# Autodesk Inventor assembly: Demonstrator
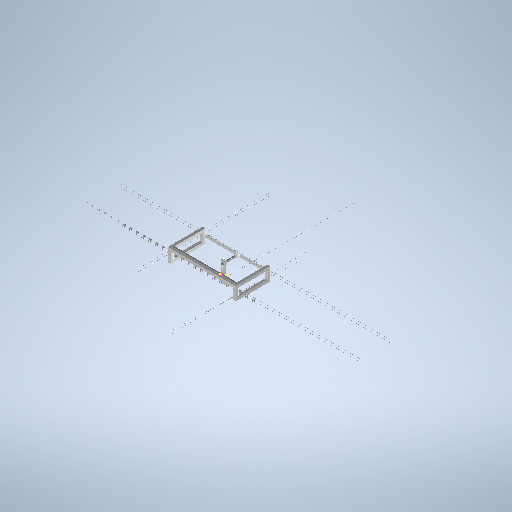
[picture p0: Inventor's stored thumbnail of the model, 512x512]
Saved by Autodesk Inventor 2025 (Build 290162010, 162A)
## iProperties
Created: 2024-11-07
Part Number: Demonstrator
Document SubType Name: Assembly
Designer: Admin
Mass: 19761.8 g
Surface Area: 23870.2 cm^2
Volume: 8041.77 cm^3
Density: 2.4574 g/cm^3
dummerWinkel: 1.5
Author: Admin
## Documents named in this file (23)
- C:\Users\Admin\Documents\Inventor\Krandemonstrator\Demonstrator.iam
- C:\Users\Admin\Documents\Inventor\Krandemonstrator\Träger.ipt
- C:\Users\Admin\Documents\Inventor\Content Center Files\R2025\de-DE\GB 798-88\Eye bolt GB 798 M4 x 20.ipt
- C:\Users\Admin\Documents\Inventor\Content Center Files\R2025\de-DE\AS 1112 (2)\AS 1112 - M4  Typ 5.ipt
- C:\Users\Admin\Documents\Inventor\Krandemonstrator\MontageAufnahmeLO.ipt
- C:\Users\Admin\Documents\Inventor\Krandemonstrator\MontageAufnahmeLOV.ipt
- C:\Users\Admin\Documents\Inventor\Krandemonstrator\FrameSide.ipt
- C:\Users\Admin\Documents\Inventor\Krandemonstrator\FrameSideR.ipt
- C:\Users\Admin\Documents\Inventor\Content Center Files\R2025\de-DE\AS 1427(03)\AS 1427 - M2 x 6(1).ipt
- C:\Users\Admin\Documents\Inventor\Krandemonstrator\Katze.iam
- C:\Users\Admin\Documents\Inventor\Krandemonstrator\UmlenkrolleHalterEinfach.iam
- C:\Users\Admin\Documents\Inventor\Krandemonstrator\SeilStange1m.ipt
- C:\Users\Admin\Documents\Inventor\Krandemonstrator\RollenhalterU.ipt
- C:\Users\Admin\Documents\Inventor\Krandemonstrator\UmlenkrolleHalterDoppelt.iam
- C:\Users\Admin\Documents\Inventor\Krandemonstrator\SeilatrappeHalter.ipt
- C:\Users\Admin\Documents\Inventor\Krandemonstrator\UmlenkrolleHalterDoppeltAngle.iam
- C:\Users\Admin\Documents\Inventor\Krandemonstrator\UmlenkrolleHalterEinfachAngle.iam
- C:\Users\Admin\Documents\Inventor\Krandemonstrator\UmlenkrolleHalterEinfachAngleB.iam
- C:\Users\Admin\Documents\Inventor\Krandemonstrator\seilatrappeHalterMini.ipt
- C:\Users\Admin\Documents\Inventor\Content Center Files\R2025\de-DE\AS 1421(4)\AS 1421 - M4 x 8 Kegelstumpf.ipt
- C:\Users\Admin\Documents\Inventor\Krandemonstrator\Schlitten.iam
- C:\Users\Admin\Documents\Inventor\Krandemonstrator\WS_10_40_930_2\WS_10_40_930_2.iam
- C:\Users\Admin\Documents\Inventor\Krandemonstrator\Bremsbelag.ipt
## Components (76 placed, 25 different names)
1. Katze:1 [sub-assembly] — KatzeLagerHO, KatzeLagerVV, KatzeSeilMutterVL, KatzeSeilMutterHL, KatzeSeilMutterVR, KatzeSeilMutterHR, KatzeSeilMutterU, KatzeSeilOeseU, KatzeGewindeSeilStumpfVL, KatzeGewindeSeilStumpfHL, KatzeGewindeSeilStumpfVR, KatzeGewindeSeilStumpfHR, KatzeSeilStumpfVL, KatzeSeilStumpfHL, KatzeSeilStumpfVR, KatzeSeilStumpfHR, Zylindrisch:83
2. Schlitten:1 [sub-assembly] — Verschiebbar:84, Zylindrisch:84, Zylindrisch:85, Zylindrisch:86, Zylindrisch:87, Planar:57, Planar:58, Planar:59, Planar:60
3. WS_10_40_930_2:1 [sub-assembly] — Starr:80, Zylindrisch:84, Zylindrisch:85, Zylindrisch:86, Zylindrisch:87
4. Bremsbelag:1 — Starr:81
5. Bremsbelag:2 — Starr:82
6. MontageAufnahmeLOVV:2 — Starr:51, SeilrolleORHscrewA, SeilrolleORHscrewB, SeilrolleORHplan
7. MontageAufnahmeLO:2 — Starr:52, SeilrolleORVplan, SeilrolleORVscrewA, SeilrolleORVscrewB
8. MontageAufnahmeLOV:1 — SeilrolleOLVAuflage, SeilrolleOLVSchraubeA, SeilrolleOLVSchraubeB
9. MontageAufnahmeLOH:1 — SeilrolleOLHAuflage, SeilrolleOLHSchraubeA, SeilrolleOLHSchraubeB
10. Träger:1 — KatzeLagerHO, KatzeLagerVV, Starr:51, Starr:52
11. FrameSide:1 — Fluchtend:1, Starr:39, SeilAtrappeHalter, Starr:80
12. FrameSideR:1 — Starr:66
13. lastseil — Verschiebbar:84, Zylindrisch:83
14. seilatrappeHalterMini:3 — SeilAtrappeHalterMini3, SeilAtrappeHalterMini3Seil
15. seilatrappeHalterMini:4 — SeilAtrappeHalterMini4, SeilAtrappeHalterMini4Seil
16. SeilStange1m:16 — SeilrolleULMVsld, SeilAtrappeHalterMini3Seil, Planar:58
17. SeilStange1m:17 — SeilrolleULMHsld, SeilAtrappeHalterMini4Seil, Planar:57
18. SeilStange1m:18 — SeilAtrappeHalterMini1Seil, SeilrolleORVver, SeilrolleURMVver
19. SeilStange1m:19 — SeilAtrappeHalterMini2Seil, SeilrolleORHver, SeilrolleURMHver
20. seilatrappeHalterMini:1 — SeilAtrappeHalterMini1, SeilAtrappeHalterMini1Seil
21. seilatrappeHalterMini:2 — SeilAtrappeHalterMini2, SeilAtrappeHalterMini2Seil
22. SeilStange1m:13 — SeilrolleURHsld, Planar:59
23. SeilStange1m:12 — SeilrolleURVsld, Planar:60
24. SeilatrappeHalter:1 — Fluchtend:1, SeilAtrappeHalterSeilA, SeilAtrappeHalterSeilB, SeilAtrappeHalter
25. SeilStange1m:1 — KatzeGewindeSeilStumpfVL, SeilrolleOLVhor
26. SeilStange1m:3 — SeilrolleOLHhor, KatzeSeilStumpfHL
27. SeilStange1m:4 — SeilrolleORHhor, KatzeSeilStumpfHR
28. SeilStange1m:5 — SeilrolleORVhor, KatzeSeilStumpfVR
29. SeilStange1m:8 — SeilAtrappeHalterSeilB, SeilrolleOLHver, SeilrolleULHver
30. SeilStange1m:9 — SeilAtrappeHalterSeilA, SeilrolleOLVver, SeilrolleULVver
31. SeilStange1m:10 — Zylindrisch:15, SeilrolleULHhor, SeilrolleURHhor
32. SeilStange1m:11 — Zylindrisch:16, SeilrolleULVhor, SeilrolleURVhor
33. SeilStange1m:14 — SeilAtrappeRollenhalterSeilB, SeilrolleULMHhor, SeilrolleURMHhor
34. SeilStange1m:15 — SeilAtrappeRollenhalterSeilA, SeilrolleULMVhor, SeilrolleURMVhor
35. AS 1427 - Metrisch M2 x 6:2 — SeilrolleOLVSchraube2, SeilrolleOLVSchraubeA
36. AS 1427 - Metrisch M2 x 6:1 — SeilrolleOLVSchraube1, SeilrolleOLVSchraubeB
37. UmlenkrolleHalterEinfach:1 [sub-assembly] — SeilrolleOLVSchraube1, SeilrolleOLVAuflage, SeilrolleOLVSchraube2, SeilrolleOLVhor, SeilrolleOLVver
38. AS 1427 - Metrisch M2 x 6:3 — SeilrolleOLHSchraube1, SeilrolleOLHSchraubeA
39. AS 1427 - Metrisch M2 x 6:4 — SeilrolleOLHSchraube2, SeilrolleOLHSchraubeB
40. UmlenkrolleHalterEinfach:2 [sub-assembly] — SeilrolleOLHSchraube1, SeilrolleOLHSchraube2, SeilrolleOLHAuflage, SeilrolleOLHhor, SeilrolleOLHver
41. AS 1112 (2) - Metrisch M4  Typ 5:4 — KatzeSeilMutterVR
42. AS 1112 (2) - Metrisch M4  Typ 5:3 — KatzeSeilMutterVL
43. AS 1112 (2) - Metrisch M4  Typ 5:2 — KatzeSeilMutterHR
44. AS 1112 (2) - Metrisch M4  Typ 5:1 — KatzeSeilMutterHL
45. AS 1112 (2) - Metrisch M4  Typ 5:5 — KatzeSeilMutterU
46. AS 1421 Kegelstumpf - Metrisch M4 x 8 Kegelstumpf:4 — KatzeGewindeSeilStumpfHR
47. AS 1421 Kegelstumpf - Metrisch M4 x 8 Kegelstumpf:1 — KatzeGewindeSeilStumpfVR
48. AS 1421 Kegelstumpf - Metrisch M4 x 8 Kegelstumpf:2 — KatzeSeilStumpfVL
49. AS 1421 Kegelstumpf - Metrisch M4 x 8 Kegelstumpf:3 — KatzeGewindeSeilStumpfHL
50. Bolt GB/T 798-1988 M4 x 20:1 — KatzeSeilOeseU
51. UmlenkrolleHalterEinfachAngle:1 [sub-assembly] — SeilrolleORVscrewAfix, SeilrolleORVscrewBfix, SeilrolleORVplan, SeilrolleORVhor, SeilrolleORVver, SeilAtrappeHalterMini1
52. AS 1427 - Metrisch M2 x 6:17 — SeilrolleORVscrewBfix, SeilrolleORVscrewB
53. AS 1427 - Metrisch M2 x 6:18 — SeilrolleORVscrewAfix, SeilrolleORVscrewA
54. AS 1427 - Metrisch M2 x 6:19 — SeilrolleORHscrewB, SeilrolleORHscrewBfix
55. AS 1427 - Metrisch M2 x 6:20 — SeilrolleORHscrewA, SeilrolleORHscrewAfix
56. UmlenkrolleHalterEinfachAngleB:1 [sub-assembly] — SeilrolleORHplan, SeilrolleORHscrewAfix, SeilrolleORHscrewBfix, SeilAtrappeHalterMini2, SeilrolleORHhor, SeilrolleORHver
57. RollenhalterU:1 — Planar:24, Zylindrisch:5, Zylindrisch:6, Planar:25, Zylindrisch:7, Zylindrisch:8, Planar:40, Zylindrisch:9, Zylindrisch:10, Starr:39, Zylindrisch:15, Zylindrisch:16, Starr:82
58. UmlenkrolleHalterDoppelt:1 [sub-assembly] — Planar:24, Starr:33, Starr:34, SeilrolleULMHhor, SeilrolleULMVhor, SeilrolleULMHsld, SeilrolleULMVsld, SeilAtrappeHalterMini3, SeilAtrappeHalterMini4
59. UmlenkrolleHalterEinfach:3 [sub-assembly] — Starr:35, Starr:36, Planar:25, SeilrolleULVver, SeilrolleULVhor
60. UmlenkrolleHalterEinfach:4 [sub-assembly] — Starr:37, Starr:38, Planar:40, SeilrolleULHver, SeilrolleULHhor
61. AS 1427 - Metrisch M2 x 6:5 — Starr:38, Zylindrisch:9
62. AS 1427 - Metrisch M2 x 6:6 — Starr:37, Zylindrisch:10
63. AS 1427 - Metrisch M2 x 6:7 — Starr:34, Zylindrisch:6
64. AS 1427 - Metrisch M2 x 6:8 — Starr:33, Zylindrisch:5
65. AS 1427 - Metrisch M2 x 6:9 — Starr:35, Zylindrisch:8
66. AS 1427 - Metrisch M2 x 6:10 — Starr:36, Zylindrisch:7
67. UmlenkrolleHalterEinfach:5 [sub-assembly] — Starr:45, Starr:44, Planar:42, SeilrolleURVhor, SeilrolleURVsld
68. UmlenkrolleHalterEinfach:6 [sub-assembly] — Starr:46, Starr:47, Planar:43, SeilrolleURHhor, SeilrolleURHsld
69. UmlenkrolleHalterDoppeltAngle:1 [sub-assembly] — Planar:54, Starr:53, Starr:54, SeilrolleURMHhor, SeilrolleURMVhor, SeilrolleURMVver, SeilrolleURMHver
70. AS 1427 - Metrisch M2 x 6:11 — Starr:47, Zylindrisch:22
71. AS 1427 - Metrisch M2 x 6:12 — Starr:46, Zylindrisch:21
72. AS 1427 - Metrisch M2 x 6:13 — Starr:45, Zylindrisch:20
73. AS 1427 - Metrisch M2 x 6:14 — Zylindrisch:18, Starr:53
74. AS 1427 - Metrisch M2 x 6:15 — Zylindrisch:17, Starr:54
75. AS 1427 - Metrisch M2 x 6:16 — Starr:44, Zylindrisch:19
76. RollenhalterU:2 — Starr:66, Zylindrisch:17, Zylindrisch:18, Planar:42, Zylindrisch:19, Zylindrisch:20, Planar:43, Zylindrisch:21, Zylindrisch:22, Planar:54, SeilAtrappeRollenhalterSeilB, SeilAtrappeRollenhalterSeilA, Starr:81
## Relationships (123: WeldJoint 46, CylindricalJoint 35, RelateRotateTranslate 24, PlanarJoint 16, Flush 1, TranslationJoint 1)
- KatzeLagerHO [PlanarJoint] (0.05 mm): Katze:1 ↔ Träger:1
- KatzeLagerVV [PlanarJoint] (0.05 mm): Katze:1 ↔ Träger:1
- KatzeSeilMutterVL [WeldJoint]: Katze:1 ↔ AS 1112 (2) - Metrisch M4  Typ 5:3
- KatzeSeilMutterHL [WeldJoint]: Katze:1 ↔ AS 1112 (2) - Metrisch M4  Typ 5:1
- KatzeSeilMutterVR [WeldJoint]: Katze:1 ↔ AS 1112 (2) - Metrisch M4  Typ 5:4
- KatzeSeilMutterHR [WeldJoint]: Katze:1 ↔ AS 1112 (2) - Metrisch M4  Typ 5:2
- KatzeSeilMutterU [WeldJoint]: Katze:1 ↔ AS 1112 (2) - Metrisch M4  Typ 5:5
- KatzeSeilOeseU [WeldJoint]: Katze:1 ↔ Bolt GB/T 798-1988 M4 x 20:1
- KatzeGewindeSeilStumpfVL [WeldJoint]: Katze:1 ↔ SeilStange1m:1
- KatzeGewindeSeilStumpfHL [WeldJoint]: Katze:1 ↔ AS 1421 Kegelstumpf - Metrisch M4 x 8 Kegelstumpf:3
- KatzeGewindeSeilStumpfVR [WeldJoint]: Katze:1 ↔ AS 1421 Kegelstumpf - Metrisch M4 x 8 Kegelstumpf:1
- KatzeGewindeSeilStumpfHR [WeldJoint]: Katze:1 ↔ AS 1421 Kegelstumpf - Metrisch M4 x 8 Kegelstumpf:4
- KatzeSeilStumpfVL [WeldJoint]: Katze:1 ↔ AS 1421 Kegelstumpf - Metrisch M4 x 8 Kegelstumpf:2
- KatzeSeilStumpfHL [WeldJoint]: Katze:1 ↔ SeilStange1m:3
- KatzeSeilStumpfVR [WeldJoint]: Katze:1 ↔ SeilStange1m:5
- KatzeSeilStumpfHR [WeldJoint]: Katze:1 ↔ SeilStange1m:4
- SeilrolleOLVSchraube1 [WeldJoint]: AS 1427 - Metrisch M2 x 6:1 ↔ UmlenkrolleHalterEinfach:1
- SeilrolleOLVSchraube2 [WeldJoint]: AS 1427 - Metrisch M2 x 6:2 ↔ UmlenkrolleHalterEinfach:1
- SeilrolleOLVAuflage [PlanarJoint]: MontageAufnahmeLOV:1 ↔ UmlenkrolleHalterEinfach:1
- SeilrolleOLVSchraubeA [CylindricalJoint]: MontageAufnahmeLOV:1 ↔ AS 1427 - Metrisch M2 x 6:2
- SeilrolleOLVSchraubeB [CylindricalJoint]: MontageAufnahmeLOV:1 ↔ AS 1427 - Metrisch M2 x 6:1
- SeilrolleOLVhor [RelateRotateTranslate] (9 mm): SeilStange1m:1 ↔ UmlenkrolleHalterEinfach:1
- SeilrolleOLVver [RelateRotateTranslate] (9 mm): SeilStange1m:9 ↔ UmlenkrolleHalterEinfach:1
- SeilrolleOLHSchraube1 [WeldJoint]: AS 1427 - Metrisch M2 x 6:3 ↔ UmlenkrolleHalterEinfach:2
- SeilrolleOLHSchraube2 [WeldJoint]: AS 1427 - Metrisch M2 x 6:4 ↔ UmlenkrolleHalterEinfach:2
- SeilrolleOLHAuflage [PlanarJoint]: MontageAufnahmeLOH:1 ↔ UmlenkrolleHalterEinfach:2
- SeilrolleOLHSchraubeA [CylindricalJoint]: MontageAufnahmeLOH:1 ↔ AS 1427 - Metrisch M2 x 6:3
- SeilrolleOLHSchraubeB [CylindricalJoint]: MontageAufnahmeLOH:1 ↔ AS 1427 - Metrisch M2 x 6:4
- SeilrolleOLHhor [RelateRotateTranslate] (9 mm): SeilStange1m:3 ↔ UmlenkrolleHalterEinfach:2
- SeilrolleOLHver [RelateRotateTranslate] (9 mm): SeilStange1m:8 ↔ UmlenkrolleHalterEinfach:2
- Planar:24: RollenhalterU:1 ↔ UmlenkrolleHalterDoppelt:1
- Starr:33 [WeldJoint]: UmlenkrolleHalterDoppelt:1 ↔ AS 1427 - Metrisch M2 x 6:8
- Starr:34 [WeldJoint]: UmlenkrolleHalterDoppelt:1 ↔ AS 1427 - Metrisch M2 x 6:7
- Zylindrisch:5 [CylindricalJoint]: RollenhalterU:1 ↔ AS 1427 - Metrisch M2 x 6:8
- Zylindrisch:6 [CylindricalJoint]: RollenhalterU:1 ↔ AS 1427 - Metrisch M2 x 6:7
- Starr:35 [WeldJoint]: UmlenkrolleHalterEinfach:3 ↔ AS 1427 - Metrisch M2 x 6:9
- Starr:36 [WeldJoint]: UmlenkrolleHalterEinfach:3 ↔ AS 1427 - Metrisch M2 x 6:10
- Planar:25: RollenhalterU:1 ↔ UmlenkrolleHalterEinfach:3
- Zylindrisch:7 [CylindricalJoint]: RollenhalterU:1 ↔ AS 1427 - Metrisch M2 x 6:10
- Zylindrisch:8 [CylindricalJoint]: RollenhalterU:1 ↔ AS 1427 - Metrisch M2 x 6:9
- Starr:37 [WeldJoint]: UmlenkrolleHalterEinfach:4 ↔ AS 1427 - Metrisch M2 x 6:6
- Starr:38 [WeldJoint]: UmlenkrolleHalterEinfach:4 ↔ AS 1427 - Metrisch M2 x 6:5
- Planar:40: RollenhalterU:1 ↔ UmlenkrolleHalterEinfach:4
- Zylindrisch:9 [CylindricalJoint]: RollenhalterU:1 ↔ AS 1427 - Metrisch M2 x 6:5
- Zylindrisch:10 [CylindricalJoint]: RollenhalterU:1 ↔ AS 1427 - Metrisch M2 x 6:6
- Fluchtend:1 [Flush]: FrameSide:1 ↔ SeilatrappeHalter:1
- SeilAtrappeHalterSeilA [CylindricalJoint]: SeilatrappeHalter:1 ↔ SeilStange1m:9
- SeilAtrappeHalterSeilB [CylindricalJoint]: SeilatrappeHalter:1 ↔ SeilStange1m:8
- Starr:39 [WeldJoint]: FrameSide:1 ↔ RollenhalterU:1
- SeilAtrappeHalter [WeldJoint]: FrameSide:1 ↔ SeilatrappeHalter:1
- Zylindrisch:15 [CylindricalJoint]: SeilStange1m:10 ↔ RollenhalterU:1
- Zylindrisch:16 [CylindricalJoint]: SeilStange1m:11 ↔ RollenhalterU:1
- SeilrolleULVver [RelateRotateTranslate] (9 mm): SeilStange1m:9 ↔ UmlenkrolleHalterEinfach:3
- SeilrolleULHver [RelateRotateTranslate] (9 mm): SeilStange1m:8 ↔ UmlenkrolleHalterEinfach:4
- SeilrolleULVhor [RelateRotateTranslate] (9 mm): SeilStange1m:11 ↔ UmlenkrolleHalterEinfach:3
- SeilrolleULHhor [RelateRotateTranslate] (9 mm): SeilStange1m:10 ↔ UmlenkrolleHalterEinfach:4
- Starr:66 [WeldJoint]: FrameSideR:1 ↔ RollenhalterU:2
- Zylindrisch:17 [CylindricalJoint]: AS 1427 - Metrisch M2 x 6:15 ↔ RollenhalterU:2
- Zylindrisch:18 [CylindricalJoint]: AS 1427 - Metrisch M2 x 6:14 ↔ RollenhalterU:2
- Starr:45 [WeldJoint]: UmlenkrolleHalterEinfach:5 ↔ AS 1427 - Metrisch M2 x 6:13
- Starr:44 [WeldJoint]: UmlenkrolleHalterEinfach:5 ↔ AS 1427 - Metrisch M2 x 6:16
- Planar:42: UmlenkrolleHalterEinfach:5 ↔ RollenhalterU:2
- Zylindrisch:19 [CylindricalJoint]: AS 1427 - Metrisch M2 x 6:16 ↔ RollenhalterU:2
- Zylindrisch:20 [CylindricalJoint]: AS 1427 - Metrisch M2 x 6:13 ↔ RollenhalterU:2
- Starr:46 [WeldJoint]: UmlenkrolleHalterEinfach:6 ↔ AS 1427 - Metrisch M2 x 6:12
- Starr:47 [WeldJoint]: UmlenkrolleHalterEinfach:6 ↔ AS 1427 - Metrisch M2 x 6:11
- Planar:43: UmlenkrolleHalterEinfach:6 ↔ RollenhalterU:2
- Zylindrisch:21 [CylindricalJoint]: AS 1427 - Metrisch M2 x 6:12 ↔ RollenhalterU:2
- Zylindrisch:22 [CylindricalJoint]: AS 1427 - Metrisch M2 x 6:11 ↔ RollenhalterU:2
- SeilrolleURHhor [RelateRotateTranslate] (9 mm): SeilStange1m:10 ↔ UmlenkrolleHalterEinfach:6
- SeilrolleURVhor [RelateRotateTranslate] (9 mm): SeilStange1m:11 ↔ UmlenkrolleHalterEinfach:5
- SeilrolleURVsld [RelateRotateTranslate] (9 mm): SeilStange1m:12 ↔ UmlenkrolleHalterEinfach:5
- SeilrolleURHsld [RelateRotateTranslate] (9 mm): SeilStange1m:13 ↔ UmlenkrolleHalterEinfach:6
- Starr:51 [WeldJoint]: MontageAufnahmeLOVV:2 ↔ Träger:1
- Starr:52 [WeldJoint]: MontageAufnahmeLO:2 ↔ Träger:1
- Planar:54: UmlenkrolleHalterDoppeltAngle:1 ↔ RollenhalterU:2
- Starr:53 [WeldJoint]: UmlenkrolleHalterDoppeltAngle:1 ↔ AS 1427 - Metrisch M2 x 6:14
- Starr:54 [WeldJoint]: UmlenkrolleHalterDoppeltAngle:1 ↔ AS 1427 - Metrisch M2 x 6:15
- SeilrolleORVscrewAfix [WeldJoint]: UmlenkrolleHalterEinfachAngle:1 ↔ AS 1427 - Metrisch M2 x 6:18
- SeilrolleORVscrewBfix [WeldJoint]: UmlenkrolleHalterEinfachAngle:1 ↔ AS 1427 - Metrisch M2 x 6:17
- SeilrolleORVplan [PlanarJoint]: MontageAufnahmeLO:2 ↔ UmlenkrolleHalterEinfachAngle:1
- SeilrolleORVscrewA [CylindricalJoint]: MontageAufnahmeLO:2 ↔ AS 1427 - Metrisch M2 x 6:18
- SeilrolleORVscrewB [CylindricalJoint]: MontageAufnahmeLO:2 ↔ AS 1427 - Metrisch M2 x 6:17
- SeilrolleORHscrewA [CylindricalJoint]: MontageAufnahmeLOVV:2 ↔ AS 1427 - Metrisch M2 x 6:20
- SeilrolleORHscrewB [CylindricalJoint]: MontageAufnahmeLOVV:2 ↔ AS 1427 - Metrisch M2 x 6:19
- SeilrolleORHplan [PlanarJoint]: MontageAufnahmeLOVV:2 ↔ UmlenkrolleHalterEinfachAngleB:1
- SeilrolleORHscrewAfix [WeldJoint]: AS 1427 - Metrisch M2 x 6:20 ↔ UmlenkrolleHalterEinfachAngleB:1
- SeilrolleORHscrewBfix [WeldJoint]: AS 1427 - Metrisch M2 x 6:19 ↔ UmlenkrolleHalterEinfachAngleB:1
- SeilAtrappeRollenhalterSeilB [CylindricalJoint]: SeilStange1m:14 ↔ RollenhalterU:2
- SeilAtrappeRollenhalterSeilA [CylindricalJoint]: SeilStange1m:15 ↔ RollenhalterU:2
- SeilrolleORHhor [RelateRotateTranslate] (9 mm): SeilStange1m:4 ↔ UmlenkrolleHalterEinfachAngleB:1
- SeilrolleORVhor [RelateRotateTranslate] (9 mm): SeilStange1m:5 ↔ UmlenkrolleHalterEinfachAngle:1
- SeilrolleORHver [RelateRotateTranslate] (9 mm): SeilStange1m:19 ↔ UmlenkrolleHalterEinfachAngleB:1
- SeilrolleORVver [RelateRotateTranslate] (9 mm): SeilStange1m:18 ↔ UmlenkrolleHalterEinfachAngle:1
- SeilrolleURMHhor [RelateRotateTranslate] (9 mm): SeilStange1m:14 ↔ UmlenkrolleHalterDoppeltAngle:1
- SeilrolleURMVhor [RelateRotateTranslate] (9 mm): SeilStange1m:15 ↔ UmlenkrolleHalterDoppeltAngle:1
- SeilrolleURMVver [RelateRotateTranslate] (9 mm): SeilStange1m:18 ↔ UmlenkrolleHalterDoppeltAngle:1
- SeilrolleURMHver [RelateRotateTranslate] (9 mm): SeilStange1m:19 ↔ UmlenkrolleHalterDoppeltAngle:1
- SeilrolleULMHhor [RelateRotateTranslate] (9 mm): SeilStange1m:14 ↔ UmlenkrolleHalterDoppelt:1
- SeilrolleULMVhor [RelateRotateTranslate] (9 mm): SeilStange1m:15 ↔ UmlenkrolleHalterDoppelt:1
- SeilrolleULMHsld [RelateRotateTranslate] (9 mm): SeilStange1m:17 ↔ UmlenkrolleHalterDoppelt:1
- SeilrolleULMVsld [RelateRotateTranslate] (9 mm): SeilStange1m:16 ↔ UmlenkrolleHalterDoppelt:1
- SeilAtrappeHalterMini1 [WeldJoint]: seilatrappeHalterMini:1 ↔ UmlenkrolleHalterEinfachAngle:1
- SeilAtrappeHalterMini1Seil [CylindricalJoint]: SeilStange1m:18 ↔ seilatrappeHalterMini:1
- SeilAtrappeHalterMini2 [WeldJoint]: seilatrappeHalterMini:2 ↔ UmlenkrolleHalterEinfachAngleB:1
- SeilAtrappeHalterMini2Seil [CylindricalJoint]: SeilStange1m:19 ↔ seilatrappeHalterMini:2
- SeilAtrappeHalterMini3 [WeldJoint]: seilatrappeHalterMini:3 ↔ UmlenkrolleHalterDoppelt:1
- SeilAtrappeHalterMini3Seil [CylindricalJoint]: seilatrappeHalterMini:3 ↔ SeilStange1m:16
- SeilAtrappeHalterMini4 [WeldJoint]: seilatrappeHalterMini:4 ↔ UmlenkrolleHalterDoppelt:1
- SeilAtrappeHalterMini4Seil [CylindricalJoint]: seilatrappeHalterMini:4 ↔ SeilStange1m:17
- Verschiebbar:84 [TranslationJoint]: Schlitten:1 ↔ lastseil
- Zylindrisch:83 [CylindricalJoint]: Katze:1 ↔ lastseil
- Starr:80 [WeldJoint] (0.2 mm): WS_10_40_930_2:1 ↔ FrameSide:1
- Zylindrisch:84 [CylindricalJoint]: Schlitten:1 ↔ WS_10_40_930_2:1
- Zylindrisch:85 [CylindricalJoint]: Schlitten:1 ↔ WS_10_40_930_2:1
- Zylindrisch:86 [CylindricalJoint]: Schlitten:1 ↔ WS_10_40_930_2:1
- Zylindrisch:87 [CylindricalJoint]: Schlitten:1 ↔ WS_10_40_930_2:1
- Planar:57: Schlitten:1 ↔ SeilStange1m:17
- Planar:58: Schlitten:1 ↔ SeilStange1m:16
- Planar:59: Schlitten:1 ↔ SeilStange1m:13
- Planar:60: Schlitten:1 ↔ SeilStange1m:12
- Starr:81 [WeldJoint]: Bremsbelag:1 ↔ RollenhalterU:2
- Starr:82 [WeldJoint]: Bremsbelag:2 ↔ RollenhalterU:1
## Named parameters: Finish2_Area = 2136.28, Finish3_Area = 43.5425, Finish4_Area = 0.0628319
note: some values were not read from the file. Shown as the stored number, unit unknown: "Finish2_Area", "Finish3_Area", "Finish4_Area".
